# Autodesk Inventor assembly: ToolHeadAssy
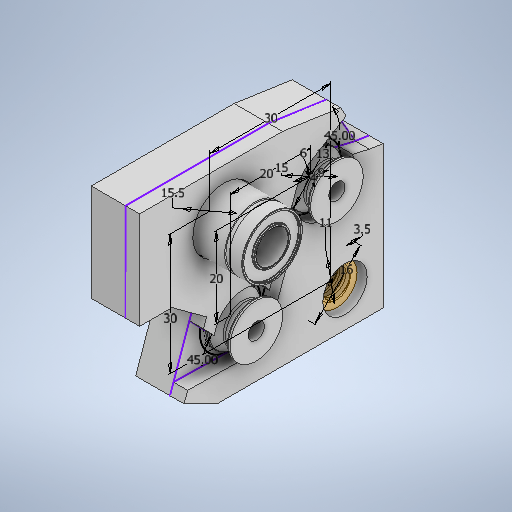
[picture p0: Inventor's stored thumbnail of the model, 512x512]
Saved by Autodesk Inventor 2025.3 (Build 293356030, 356C)
## iProperties
Created: 2025-10-22
Part Number: ToolHeadAssy
Document SubType Name: Assembly
Designer: tvoko
Author: tvoko
## Documents named in this file (5)
- C:\Users\tvoko\Github\DIY-Coil-Winder\CAD\ToolHeadAssy.iam
- C:\Users\tvoko\Github\DIY-Coil-Winder\CAD\Imports\NEMA 17 Stepper Motor 39mm-NEMA 17 Stepper Motor 39mm\T8 Nut 1.5\T8 Nut 1.5.ipt
- **C:\Users\tvoko\Github\DIY-Coil-Winder\CAD\Main.iam*LocalDocs*xAaaaqkbaAaaaaaaaAaaaakp3Be*3.Linear Bearing-LM8UU.ipt
- C:\Users\tvoko\Github\DIY-Coil-Winder\CAD\GuideBlock.ipt
- C:\Users\tvoko\Github\DIY-Coil-Winder\CAD\Imports\uxcell_V624ZZ_4mmx13mmx6mm.ipt
## Components (5 placed, 4 different names)
1. T8 Nut 1.5:1 — Mate:4, Mate:5, Mate:6
2. 3.Linear Bearing-LM8UU:1 — Mate:1, Mate:7
3. GuideBlock:1 — Mate:1, Mate:2, Mate:3, Mate:4, Mate:5, Mate:6, Mate:7, Mate:8, Mate:9
4. uxcell_V624ZZ_4mmx13mmx6mm:1 — Mate:3, Mate:9
5. uxcell_V624ZZ_4mmx13mmx6mm:2 — Mate:2, Mate:8
## Relationships (9: Mate 9)
- Mate:1: 3.Linear Bearing-LM8UU:1 ↔ GuideBlock:1
- Mate:2: GuideBlock:1 ↔ uxcell_V624ZZ_4mmx13mmx6mm:2
- Mate:3: GuideBlock:1 ↔ uxcell_V624ZZ_4mmx13mmx6mm:1
- Mate:4: T8 Nut 1.5:1 ↔ GuideBlock:1
- Mate:5: T8 Nut 1.5:1 ↔ GuideBlock:1
- Mate:6: T8 Nut 1.5:1 ↔ GuideBlock:1
- Mate:7: 3.Linear Bearing-LM8UU:1 ↔ GuideBlock:1
- Mate:8: GuideBlock:1 ↔ uxcell_V624ZZ_4mmx13mmx6mm:2
- Mate:9: GuideBlock:1 ↔ uxcell_V624ZZ_4mmx13mmx6mm:1
